# Autodesk Inventor assembly: UpperArmLeft
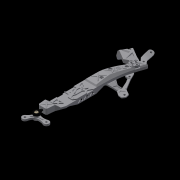
[picture p0: Inventor's stored thumbnail of the model, 180x180]
Saved by Autodesk Inventor 2020 (Build 240168000, 168)
## iProperties
Created: 2016-10-01
Part Number: UpperArmLeft
Document SubType Name: Assembly
Designer: Val
Author: Val
## Documents named in this file (7)
- C:\Users\valer\Desktop\elysium-max-exoskeleton\src\Assemblies\UpperArmLeft.iam
- C:\Users\valer\Desktop\elysium-max-exoskeleton\src\UpperArmLeft.ipt
- C:\Users\valer\Desktop\elysium-max-exoskeleton\src\UpperArmShoulderLeft.ipt
- C:\Users\valer\Desktop\elysium-max-exoskeleton\src\UpperArmTricepLeft.ipt
- C:\Users\valer\Desktop\elysium-max-exoskeleton\src\External\Bearing.iam
- C:\Users\valer\Desktop\elysium-max-exoskeleton\src\UpperArmConnectorLeft.ipt
- C:\Users\valer\Desktop\elysium-max-exoskeleton\src\ElbowSubConnector.ipt
## Components (6 placed, 6 different names)
1. UpperArmLeft:1 — Mate:4, Mate:5, Mate:6, Mate:7, Flush:1, Angle:1, Mate:8, Mate:9, Flush:2, Mate:12, Mate:13, Mate:14
2. UpperArmShoulderLeft:1 — Mate:12, Mate:13, Mate:14
3. UpperArmTricepLeft:1 — Mate:4, Mate:5, Mate:6
4. Bearing:1 [sub-assembly] — Mate:7, Flush:1, Angle:1, Mate:8, Mate:10, Mate:11
5. UpperArmTwistConnectorLeft:1 — Mate:9, Flush:2
6. ElbowSubConnectorLeft:1 — Mate:10, Mate:11
## Relationships (14: Mate 11, Flush 2, Angle 1)
- Mate:4: UpperArmLeft:1 ↔ UpperArmTricepLeft:1
- Mate:5: UpperArmLeft:1 ↔ UpperArmTricepLeft:1
- Mate:6: UpperArmLeft:1 ↔ UpperArmTricepLeft:1
- Mate:7: UpperArmLeft:1 ↔ Bearing:1
- Flush:1 (-15 mm): UpperArmLeft:1 ↔ Bearing:1
- Angle:1 (0 deg): UpperArmLeft:1 ↔ Bearing:1
- Mate:8 (-15 mm): UpperArmLeft:1 ↔ Bearing:1
- Mate:9: UpperArmLeft:1 ↔ UpperArmTwistConnectorLeft:1
- Flush:2: UpperArmLeft:1 ↔ UpperArmTwistConnectorLeft:1
- Mate:10: Bearing:1 ↔ ElbowSubConnectorLeft:1
- Mate:11: Bearing:1 ↔ ElbowSubConnectorLeft:1
- Mate:12: UpperArmLeft:1 ↔ UpperArmShoulderLeft:1
- Mate:13: UpperArmLeft:1 ↔ UpperArmShoulderLeft:1
- Mate:14: UpperArmLeft:1 ↔ UpperArmShoulderLeft:1
